# Autodesk Inventor assembly: 固定robot_hand
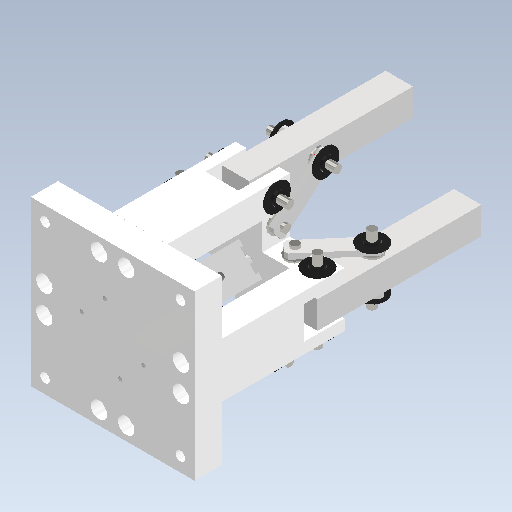
[picture p0: Inventor's stored thumbnail of the model, 512x512]
Saved by Autodesk Inventor 2021 (Build 250183000, 183)
## iProperties
Created: 2021-10-23
Part Number: 固定robot_hand
Document SubType Name: Assembly
Designer: ryusei
Author: ryusei
## Documents named in this file (16)
- C:\Users\ryusei\Documents\Inventor\robot_design3\完成版\固定robot_hand.iam
- C:\Users\ryusei\Documents\Inventor\robot_design3\完成版\部品\ハンド土台.ipt
- C:\Users\ryusei\Documents\Inventor\robot_design3\完成版\部品\ハンド支え.ipt
- C:\Users\ryusei\Documents\Inventor\robot_design3\完成版\部品\シリンダ固定.ipt
- C:\Users\ryusei\Documents\Inventor\robot_design3\完成版\部品\MBDA6×15_シリンダコガネイ\伸びるやつ１.ipt
- C:\Users\ryusei\Documents\Inventor\robot_design3\完成版\部品\MBDA6×15_シリンダコガネイ\伸びるやつ2.ipt
- C:\Users\ryusei\Documents\Inventor\robot_design3\完成版\部品\MBDA6×15_シリンダコガネイ\本体.ipt
- C:\Users\ryusei\Documents\Inventor\robot_design3\完成版\部品\シリンダ先端パーツ.ipt
- C:\Users\ryusei\Documents\Inventor\robot_design3\完成版\部品\ステンレス平行ピンΦ3h7_30.ipt
- C:\Users\ryusei\Documents\Inventor\robot_design3\完成版\部品\ハンド10×10×60.ipt
- C:\Users\ryusei\Documents\Inventor\robot_design3\完成版\部品\MF63ZZ_ベアリング.ipt
- C:\Users\ryusei\Documents\Inventor\robot_design3\完成版\部品\ステンレス平行ピンΦ3h7_25.ipt
- C:\Users\ryusei\Documents\Inventor\robot_design3\完成版\部品\ステンレス平行ピンΦ3h7_18.ipt
- C:\Users\ryusei\Documents\Inventor\robot_design3\完成版\部品\樹脂ワッシャ(ポリスライダー).ipt
- C:\Users\ryusei\Documents\Inventor\robot_design3\完成版\部品\リンク26×6×2.ipt
- C:\Users\ryusei\Documents\Inventor\robot_design3\完成版\部品\Φ3軸用プッシュナット.ipt
## Components (99 placed, 15 different names)
1. ハンド土台:1
2. ハンド支え:1
3. ハンド支え:2
4. ハンド支え:3 — 角度:2
5. ハンド支え:4
6. シリンダ固定:1
7. 伸びるやつ１:1
8. 伸びるやつ2:1
9. 本体:1
10. シリンダ固定:2
11. シリンダ先端パーツ:1
12. ステンレス平行ピンΦ3h7_30:1
13. ステンレス平行ピンΦ3h7_30:2
14. ステンレス平行ピンΦ3h7_30:3
15. ステンレス平行ピンΦ3h7_30:4
16. ハンド10×10×60:1
17. ハンド10×10×60:2
18. ハンド10×10×60:3
19. ハンド10×10×60:4 — 角度:2
20. MF63ZZ_ベアリング:1
21. MF63ZZ_ベアリング:2
22. MF63ZZ_ベアリング:3
23. MF63ZZ_ベアリング:4
24. MF63ZZ_ベアリング:5
25. MF63ZZ_ベアリング:6
26. MF63ZZ_ベアリング:7
27. MF63ZZ_ベアリング:8
28. MF63ZZ_ベアリング:9
29. MF63ZZ_ベアリング:10
30. MF63ZZ_ベアリング:11
31. MF63ZZ_ベアリング:12
32. MF63ZZ_ベアリング:13
33. MF63ZZ_ベアリング:14
34. MF63ZZ_ベアリング:15
35. MF63ZZ_ベアリング:16
36. MF63ZZ_ベアリング:17
37. MF63ZZ_ベアリング:18
38. MF63ZZ_ベアリング:19
39. MF63ZZ_ベアリング:20
40. MF63ZZ_ベアリング:21
41. MF63ZZ_ベアリング:22
42. MF63ZZ_ベアリング:23
43. MF63ZZ_ベアリング:24
44. ステンレス平行ピンΦ3h7_25:1
45. ステンレス平行ピンΦ3h7_25:2
46. ステンレス平行ピンΦ3h7_25:3
47. ステンレス平行ピンΦ3h7_25:4
48. ステンレス平行ピンΦ3h7_18:1
49. ステンレス平行ピンΦ3h7_18:2
50. ステンレス平行ピンΦ3h7_18:3
51. ステンレス平行ピンΦ3h7_18:4
52. 樹脂ワッシャ(ポリスライダー):1
53. 樹脂ワッシャ(ポリスライダー):2
54. 樹脂ワッシャ(ポリスライダー):3
55. 樹脂ワッシャ(ポリスライダー):4
56. 樹脂ワッシャ(ポリスライダー):5
57. 樹脂ワッシャ(ポリスライダー):6
58. 樹脂ワッシャ(ポリスライダー):7
59. 樹脂ワッシャ(ポリスライダー):8
60. 樹脂ワッシャ(ポリスライダー):9
61. 樹脂ワッシャ(ポリスライダー):10
62. 樹脂ワッシャ(ポリスライダー):11
63. 樹脂ワッシャ(ポリスライダー):12
64. 樹脂ワッシャ(ポリスライダー):13
65. 樹脂ワッシャ(ポリスライダー):14
66. 樹脂ワッシャ(ポリスライダー):15
67. 樹脂ワッシャ(ポリスライダー):16
68. 樹脂ワッシャ(ポリスライダー):17
69. 樹脂ワッシャ(ポリスライダー):18
70. 樹脂ワッシャ(ポリスライダー):19
71. 樹脂ワッシャ(ポリスライダー):20
72. 樹脂ワッシャ(ポリスライダー):21
73. 樹脂ワッシャ(ポリスライダー):22
74. 樹脂ワッシャ(ポリスライダー):23
75. 樹脂ワッシャ(ポリスライダー):24
76. リンク26×6×2:1
77. リンク26×6×2:2
78. リンク26×6×2:3
79. リンク26×6×2:4
80. リンク26×6×2:5
81. リンク26×6×2:6
82. リンク26×6×2:7
83. リンク26×6×2:8
84. Φ3軸用プッシュナット:1
85. Φ3軸用プッシュナット:2
86. Φ3軸用プッシュナット:3
87. Φ3軸用プッシュナット:4
88. Φ3軸用プッシュナット:5
89. Φ3軸用プッシュナット:6
90. Φ3軸用プッシュナット:7
91. Φ3軸用プッシュナット:8
92. Φ3軸用プッシュナット:9
93. Φ3軸用プッシュナット:10
94. Φ3軸用プッシュナット:11
95. Φ3軸用プッシュナット:12
96. Φ3軸用プッシュナット:13
97. Φ3軸用プッシュナット:14
98. Φ3軸用プッシュナット:15
99. Φ3軸用プッシュナット:16
## Relationships (117: Insert 113, Angle 2, Mate 1, CylindricalJoint 1)
- [Insert]: ハンド土台:1 ↔ ハンド支え:1
- [Insert]: ハンド土台:1 ↔ ハンド支え:1
- [Insert]: ハンド土台:1 ↔ ハンド支え:2
- [Insert]: ハンド土台:1 ↔ ハンド支え:2
- [Insert]: ハンド土台:1 ↔ ハンド支え:4
- [Insert]: ハンド土台:1 ↔ ハンド支え:4
- [Insert]: ハンド土台:1 ↔ ハンド支え:3
- [Insert]: ハンド土台:1 ↔ ハンド支え:3
- [Insert]: 伸びるやつ１:1 ↔ 伸びるやつ2:1
- [Insert]: シリンダ固定:1 ↔ 本体:1
- [Insert]: シリンダ固定:1 ↔ 本体:1
- [Insert]: 本体:1 ↔ シリンダ固定:2
- [Mate]: 伸びるやつ１:1 ↔ 本体:1
- [Insert]: 伸びるやつ2:1 ↔ シリンダ先端パーツ:1
- [Angle] (0 deg): ハンド支え:4 ↔ シリンダ先端パーツ:1
- [Insert] (-5 mm): ハンド支え:4 ↔ ステンレス平行ピンΦ3h7_30:4
- [Insert] (-5 mm): ハンド支え:2 ↔ ステンレス平行ピンΦ3h7_30:2
- [Insert] (-5 mm): ハンド支え:1 ↔ ステンレス平行ピンΦ3h7_30:1
- [Insert] (-5 mm): ハンド支え:3 ↔ ステンレス平行ピンΦ3h7_30:3
- [Insert]: ハンド10×10×60:4 ↔ MF63ZZ_ベアリング:23
- [Insert]: ハンド10×10×60:4 ↔ MF63ZZ_ベアリング:22
- [Insert]: ハンド10×10×60:4 ↔ MF63ZZ_ベアリング:24
- [Insert]: ハンド10×10×60:4 ↔ MF63ZZ_ベアリング:18
- [Insert]: シリンダ先端パーツ:1 ↔ MF63ZZ_ベアリング:3
- [Insert]: シリンダ先端パーツ:1 ↔ MF63ZZ_ベアリング:4
- [Insert]: シリンダ先端パーツ:1 ↔ MF63ZZ_ベアリング:2
- [Insert]: シリンダ先端パーツ:1 ↔ MF63ZZ_ベアリング:1
- [Insert]: シリンダ先端パーツ:1 ↔ MF63ZZ_ベアリング:7
- [Insert]: シリンダ先端パーツ:1 ↔ MF63ZZ_ベアリング:5
- [Insert]: シリンダ先端パーツ:1 ↔ MF63ZZ_ベアリング:8
- [Insert]: シリンダ先端パーツ:1 ↔ MF63ZZ_ベアリング:6
- [Insert]: ハンド10×10×60:3 ↔ MF63ZZ_ベアリング:9
- [Insert]: ハンド10×10×60:3 ↔ MF63ZZ_ベアリング:12
- [Insert]: ハンド10×10×60:2 ↔ MF63ZZ_ベアリング:10
- [Insert]: ハンド10×10×60:2 ↔ MF63ZZ_ベアリング:11
- [Insert]: ハンド10×10×60:1 ↔ MF63ZZ_ベアリング:15
- [Insert]: ハンド10×10×60:1 ↔ MF63ZZ_ベアリング:16
- [Insert]: ハンド10×10×60:3 ↔ MF63ZZ_ベアリング:17
- [Insert]: ハンド10×10×60:3 ↔ MF63ZZ_ベアリング:20
- [Insert]: ハンド10×10×60:2 ↔ MF63ZZ_ベアリング:21
- [Insert]: ハンド10×10×60:2 ↔ MF63ZZ_ベアリング:13
- [Insert]: ハンド10×10×60:1 ↔ MF63ZZ_ベアリング:19
- [Insert]: ハンド10×10×60:1 ↔ MF63ZZ_ベアリング:14
- [Insert] (9.4 mm): ステンレス平行ピンΦ3h7_30:3 ↔ MF63ZZ_ベアリング:18
- [Insert] (9.4 mm): ステンレス平行ピンΦ3h7_30:1 ↔ MF63ZZ_ベアリング:19
- [Insert] (9.4 mm): ステンレス平行ピンΦ3h7_30:2 ↔ MF63ZZ_ベアリング:12
- [Insert] (9.4 mm): ステンレス平行ピンΦ3h7_30:4 ↔ MF63ZZ_ベアリング:11
- [Insert] (-6.9 mm): MF63ZZ_ベアリング:24 ↔ ステンレス平行ピンΦ3h7_25:4
- [Insert] (-6.9 mm): MF63ZZ_ベアリング:13 ↔ ステンレス平行ピンΦ3h7_25:3
- [Insert] (-6.9 mm): MF63ZZ_ベアリング:20 ↔ ステンレス平行ピンΦ3h7_25:2
- [Insert] (-6.9 mm): MF63ZZ_ベアリング:14 ↔ ステンレス平行ピンΦ3h7_25:1
- [Insert] (-3.4 mm): MF63ZZ_ベアリング:3 ↔ ステンレス平行ピンΦ3h7_18:1
- [Insert] (-3.4 mm): MF63ZZ_ベアリング:4 ↔ ステンレス平行ピンΦ3h7_18:2
- [Insert] (-3.4 mm): MF63ZZ_ベアリング:5 ↔ ステンレス平行ピンΦ3h7_18:4
- [Insert] (-3.4 mm): MF63ZZ_ベアリング:1 ↔ ステンレス平行ピンΦ3h7_18:3
- [Insert]: MF63ZZ_ベアリング:3 ↔ 樹脂ワッシャ(ポリスライダー):12
- [Insert]: MF63ZZ_ベアリング:4 ↔ 樹脂ワッシャ(ポリスライダー):5
- [Insert]: MF63ZZ_ベアリング:1 ↔ 樹脂ワッシャ(ポリスライダー):10
- [Insert]: MF63ZZ_ベアリング:2 ↔ 樹脂ワッシャ(ポリスライダー):11
- [Insert]: MF63ZZ_ベアリング:8 ↔ 樹脂ワッシャ(ポリスライダー):9
- [Insert]: MF63ZZ_ベアリング:6 ↔ 樹脂ワッシャ(ポリスライダー):8
- [Insert]: MF63ZZ_ベアリング:5 ↔ 樹脂ワッシャ(ポリスライダー):7
- [Insert]: MF63ZZ_ベアリング:7 ↔ 樹脂ワッシャ(ポリスライダー):6
- [Insert]: MF63ZZ_ベアリング:24 ↔ 樹脂ワッシャ(ポリスライダー):1
- [Insert]: MF63ZZ_ベアリング:18 ↔ 樹脂ワッシャ(ポリスライダー):3
- [Insert]: MF63ZZ_ベアリング:23 ↔ 樹脂ワッシャ(ポリスライダー):4
- [Insert]: MF63ZZ_ベアリング:22 ↔ 樹脂ワッシャ(ポリスライダー):2
- [Insert]: MF63ZZ_ベアリング:13 ↔ 樹脂ワッシャ(ポリスライダー):16
- [Insert]: MF63ZZ_ベアリング:21 ↔ 樹脂ワッシャ(ポリスライダー):15
- [Insert]: MF63ZZ_ベアリング:11 ↔ 樹脂ワッシャ(ポリスライダー):13
- [Insert]: MF63ZZ_ベアリング:10 ↔ 樹脂ワッシャ(ポリスライダー):14
- [Insert]: MF63ZZ_ベアリング:9 ↔ 樹脂ワッシャ(ポリスライダー):19
- [Insert]: MF63ZZ_ベアリング:12 ↔ 樹脂ワッシャ(ポリスライダー):20
- [Insert]: MF63ZZ_ベアリング:20 ↔ 樹脂ワッシャ(ポリスライダー):17
- [Insert]: MF63ZZ_ベアリング:17 ↔ 樹脂ワッシャ(ポリスライダー):18
- [Insert]: MF63ZZ_ベアリング:14 ↔ 樹脂ワッシャ(ポリスライダー):23
- [Insert]: MF63ZZ_ベアリング:19 ↔ 樹脂ワッシャ(ポリスライダー):24
- [Insert]: MF63ZZ_ベアリング:15 ↔ 樹脂ワッシャ(ポリスライダー):22
- [Insert]: MF63ZZ_ベアリング:16 ↔ 樹脂ワッシャ(ポリスライダー):21
- [Insert]: 樹脂ワッシャ(ポリスライダー):19 ↔ リンク26×6×2:2
- [Insert]: 樹脂ワッシャ(ポリスライダー):23 ↔ リンク26×6×2:1
- [Insert]: 樹脂ワッシャ(ポリスライダー):1 ↔ リンク26×6×2:5
- [Insert]: 樹脂ワッシャ(ポリスライダー):16 ↔ リンク26×6×2:6
- [Insert]: 樹脂ワッシャ(ポリスライダー):17 ↔ リンク26×6×2:8
- [Insert]: 樹脂ワッシャ(ポリスライダー):22 ↔ リンク26×6×2:3
- [Insert]: 樹脂ワッシャ(ポリスライダー):14 ↔ リンク26×6×2:4
- [Insert]: 樹脂ワッシャ(ポリスライダー):2 ↔ リンク26×6×2:7
- [Insert]: 樹脂ワッシャ(ポリスライダー):5 ↔ リンク26×6×2:5
- [Insert]: 樹脂ワッシャ(ポリスライダー):6 ↔ リンク26×6×2:7
- [Insert]: 樹脂ワッシャ(ポリスライダー):7 ↔ リンク26×6×2:6
- [Insert]: 樹脂ワッシャ(ポリスライダー):9 ↔ リンク26×6×2:8
- [Insert]: 樹脂ワッシャ(ポリスライダー):10 ↔ リンク26×6×2:2
- [Insert]: 樹脂ワッシャ(ポリスライダー):11 ↔ リンク26×6×2:3
- [Insert]: 樹脂ワッシャ(ポリスライダー):12 ↔ リンク26×6×2:1
- [Insert]: 樹脂ワッシャ(ポリスライダー):8 ↔ リンク26×6×2:4
- [CylindricalJoint]: 伸びるやつ１:1 ↔ 本体:1
- [Insert]: リンク26×6×2:4 ↔ Φ3軸用プッシュナット:1
- [Insert]: ハンド支え:4 ↔ Φ3軸用プッシュナット:2
- [Insert]: リンク26×6×2:8 ↔ Φ3軸用プッシュナット:15
- [Insert]: ハンド支え:2 ↔ Φ3軸用プッシュナット:16
- [Insert]: リンク26×6×2:2 ↔ Φ3軸用プッシュナット:13
- [Insert]: ハンド支え:2 ↔ Φ3軸用プッシュナット:14
- [Insert]: リンク26×6×2:3 ↔ Φ3軸用プッシュナット:12
- [Insert]: ハンド支え:1 ↔ Φ3軸用プッシュナット:11
- [Insert]: ハンド支え:1 ↔ Φ3軸用プッシュナット:9
- [Insert]: リンク26×6×2:1 ↔ Φ3軸用プッシュナット:10
- [Insert]: ハンド支え:3 ↔ Φ3軸用プッシュナット:8
- [Insert]: リンク26×6×2:5 ↔ Φ3軸用プッシュナット:7
- [Insert]: ハンド支え:3 ↔ Φ3軸用プッシュナット:6
- [Insert]: リンク26×6×2:7 ↔ Φ3軸用プッシュナット:5
- [Insert]: リンク26×6×2:6 ↔ Φ3軸用プッシュナット:3
- [Insert]: ハンド支え:4 ↔ Φ3軸用プッシュナット:4
- [Insert]: ハンド土台:1 ↔ シリンダ固定:2
- [Insert]: ハンド土台:1 ↔ シリンダ固定:2
- [Insert]: ハンド土台:1 ↔ シリンダ固定:1
- [Insert]: ハンド土台:1 ↔ シリンダ固定:1
- 角度:2 [Angle] (0 deg): ハンド支え:3 ↔ ハンド10×10×60:4
